# Autodesk Inventor assembly: richWithHodoscope
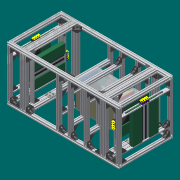
[picture p0: Inventor's stored thumbnail of the model, 180x180]
Saved by Autodesk Inventor 2016 SP1 (Build 200210100, 210)
## iProperties
Created: 2016-02-10
Part Number: richWithHodoscope
Document SubType Name: Assembly
Designer: Sawaiz
Author: Sawaiz
## Documents named in this file (4)
- C:\Users\sawaiz\oneDrive\projects\modularRichFrame\richWithHodoscope.iam
- C:\Users\sawaiz\oneDrive\projects\modularRichFrame\richInMount.iam
- C:\Users\sawaiz\OneDrive\projects\modularRICH\testMount\fingerHodoscope\hodoscopeHolder.iam
- C:\Users\sawaiz\oneDrive\projects\modularRichFrame\moduleConnectorBracket.iam
## Components (7 placed, 3 different names)
1. richInMount:1 [sub-assembly] — Mate:1, Mate:2, Flush:1, Flush:2, Flush:3, Flush:4, Flush:6, Flush:9
2. hodoscopeHolder:1 [sub-assembly] — Mate:1, Flush:3, Flush:4, Mate:3, Flush:5, Mate:5, Flush:8, Symmetry:2, Symmetry:3, Symmetry:4
3. hodoscopeHolder:2 [sub-assembly] — Mate:2, Flush:1, Flush:2, Mate:4, Symmetry:2, Symmetry:3, Symmetry:4
4. moduleConnectorBracket:1 [sub-assembly] — Mate:3, Flush:5, Flush:10, Symmetry:1, Flush:11
5. moduleConnectorBracket:2 [sub-assembly] — Mate:4, Flush:6, Flush:10, Symmetry:1
6. moduleConnectorBracket:3 [sub-assembly] — Flush:7, Flush:9
7. moduleConnectorBracket:4 [sub-assembly] — Flush:7, Mate:5, Flush:8, Flush:11
## Relationships (20: Flush 11, Mate 5, Symmetry 4)
- Mate:1: richInMount:1 ↔ hodoscopeHolder:1
- Mate:2: richInMount:1 ↔ hodoscopeHolder:2
- Flush:1: richInMount:1 ↔ hodoscopeHolder:2
- Flush:2: richInMount:1 ↔ hodoscopeHolder:2
- Flush:3: richInMount:1 ↔ hodoscopeHolder:1
- Flush:4: richInMount:1 ↔ hodoscopeHolder:1
- Mate:3: hodoscopeHolder:1 ↔ moduleConnectorBracket:1
- Flush:5 (2 mm): hodoscopeHolder:1 ↔ moduleConnectorBracket:1
- Mate:4: hodoscopeHolder:2 ↔ moduleConnectorBracket:2
- Flush:6 (2 mm): richInMount:1 ↔ moduleConnectorBracket:2
- Flush:7: moduleConnectorBracket:3 ↔ moduleConnectorBracket:4
- Mate:5: hodoscopeHolder:1 ↔ moduleConnectorBracket:4
- Flush:8 (2 mm): hodoscopeHolder:1 ↔ moduleConnectorBracket:4
- Flush:9 (2 mm): richInMount:1 ↔ moduleConnectorBracket:3
- Flush:10: moduleConnectorBracket:1 ↔ moduleConnectorBracket:2
- Symmetry:1: moduleConnectorBracket:1 ↔ moduleConnectorBracket:2
- Symmetry:2: hodoscopeHolder:1 ↔ hodoscopeHolder:2
- Symmetry:3: hodoscopeHolder:1 ↔ hodoscopeHolder:2
- Symmetry:4: hodoscopeHolder:1 ↔ hodoscopeHolder:2
- Flush:11: moduleConnectorBracket:1 ↔ moduleConnectorBracket:4
